# Autodesk Inventor assembly: E006-Carter
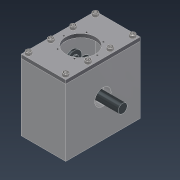
[picture p0: Inventor's stored thumbnail of the model, 180x180]
Saved by Autodesk Inventor 2021.3 (Build 253353000, 353)
## iProperties
Created: 2022-04-01
Part Number: E006-Carter
Document SubType Name: Assembly
Designer: remi
Author: remi
## Documents named in this file (5)
- C:\Users\remi\OneDrive\Documents\Cours\05-HEVS\S2fb\mechanic\CCo\project\Compressor\E006-Carter.iam
- C:\Users\remi\OneDrive\Documents\Cours\05-HEVS\S2fb\mechanic\CCo\project\Compressor\P016-Carter_corps.ipt
- C:\Users\remi\OneDrive\Documents\Cours\05-HEVS\S2fb\mechanic\CCo\project\Compressor\P015-Vilbrequin.ipt
- C:\Users\remi\OneDrive\Documents\Cours\05-HEVS\S2fb\mechanic\CCo\project\Compressor\P017-Carter_chapeau.ipt
- C:\Users\remi\OneDrive\Documents\Cours\05-HEVS\S2fb\mechanic\CCo\project\Compressor\R2021\en-US\AS 1420\AS 1420 - 1973 - M4 x 12.ipt
## Components (11 placed, 4 different names)
1. P016-Carter_corps:1 — Mate:1, Mate:2, Flush:1, Flush:2
2. P015-Vilbrequin:1 — Mate:1
3. P017-Carter_chapeau:1 — Mate:2, Flush:1, Flush:2, Insert:1, Insert:2, Insert:3, Insert:4, Insert:5, Insert:6, Insert:7, Insert:8
4. AS 1420 - Metric M4 x 12:1 — Insert:1
5. AS 1420 - Metric M4 x 12:2 — Insert:2
6. AS 1420 - Metric M4 x 12:3 — Insert:3
7. AS 1420 - Metric M4 x 12:4 — Insert:4
8. AS 1420 - Metric M4 x 12:5 — Insert:5
9. AS 1420 - Metric M4 x 12:6 — Insert:6
10. AS 1420 - Metric M4 x 12:7 — Insert:7
11. AS 1420 - Metric M4 x 12:8 — Insert:8
## Relationships (12: Insert 8, Mate 2, Flush 2)
- Mate:1: P016-Carter_corps:1 ↔ P015-Vilbrequin:1
- Mate:2: P016-Carter_corps:1 ↔ P017-Carter_chapeau:1
- Flush:1: P016-Carter_corps:1 ↔ P017-Carter_chapeau:1
- Flush:2: P016-Carter_corps:1 ↔ P017-Carter_chapeau:1
- Insert:1: P017-Carter_chapeau:1 ↔ AS 1420 - Metric M4 x 12:1
- Insert:2: P017-Carter_chapeau:1 ↔ AS 1420 - Metric M4 x 12:2
- Insert:3: P017-Carter_chapeau:1 ↔ AS 1420 - Metric M4 x 12:3
- Insert:4: P017-Carter_chapeau:1 ↔ AS 1420 - Metric M4 x 12:4
- Insert:5: P017-Carter_chapeau:1 ↔ AS 1420 - Metric M4 x 12:5
- Insert:6: P017-Carter_chapeau:1 ↔ AS 1420 - Metric M4 x 12:6
- Insert:7: P017-Carter_chapeau:1 ↔ AS 1420 - Metric M4 x 12:7
- Insert:8: P017-Carter_chapeau:1 ↔ AS 1420 - Metric M4 x 12:8
